# Autodesk Inventor assembly: ASY MSC 500 BELLY
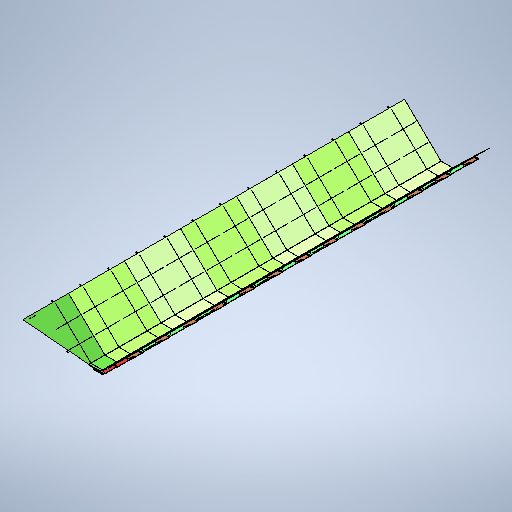
[picture p0: Inventor's stored thumbnail of the model, 512x512]
Saved by Autodesk Inventor 2025 (Build 290162010, 162A)
## iProperties
Created: 2024-07-22
Part Number: ASY MSC 500 BELLY
Document SubType Name: Assembly
Designer: pokla
Stock Number: ASY МОО 500 брюхо
Author: pokla
## Documents named in this file (7)
- C:\Users\admin\YandexDisk-badmisterfox\домашниий пк\Inventor\Manturovo\Manturovo_Se-clar\ASY MSC 204 BELLY.iam
- C:\Users\admin\YandexDisk-badmisterfox\домашниий пк\Inventor\Manturovo\Manturovo_Se-clar\MSC 501 sheet belly main.ipt
- C:\Users\admin\YandexDisk-badmisterfox\домашниий пк\Inventor\Manturovo\Manturovo_Se-clar\MSC 502 sheet belly-neck.ipt
- C:\Users\admin\YandexDisk-badmisterfox\домашниий пк\Inventor\Manturovo\Manturovo_Se-clar\MSC 504 stringer board belly.ipt
- C:\Users\admin\YandexDisk-badmisterfox\домашниий пк\Inventor\Manturovo\Manturovo_Se-clar\MSC 503 rib belly.ipt
- C:\Users\admin\YandexDisk-badmisterfox\домашниий пк\Inventor\Manturovo\Manturovo_Se-clar\MSC 505 sheet belly-neck.ipt
- C:\Users\admin\YandexDisk-badmisterfox\домашниий пк\Inventor\Manturovo\Manturovo_Se-clar\MSC 506 stringer belly short.ipt
## Components (62 placed, 7 different names)
1. MSC 501 sheet belly main:1
2. MSC 501 sheet belly main:2
3. MSC 501 sheet belly main:3
4. MSC 502 sheet belly-neck:1 — Rigid:24
5. MSC 501 sheet belly main:4
6. MSC 501 sheet belly main:5 — Rigid:23, Rigid:24
7. MSC 501 sheet belly main:6 — Mate:4, Mate:5, Mate:6, Mate:7, Flush:1, Mate:9, Mate:10, Flush:2, Mate:11, Mate:12
8. MSC 503 rib belly:1 — Rigid:17, Rigid:20, Rigid:21, Mate:13
9. MSC 503 rib belly:2 — Rigid:18, Rigid:19, Mate:11, Mate:12, Mate:13
10. MSC 504 stringer board belly:1 — Rigid:21, Flush:2
11. MSC 504 stringer board belly:2 — Rigid:20
12. MSC 504 stringer board belly:3 — Rigid:19
13. MSC 504 stringer board belly:4 — Rigid:18
14. MSC 505 sheet belly-neck:1 — Rigid:23
15. MSC 506 stringer belly short:1 — Rigid:25
16. MSC 506 stringer belly short:2 — Rigid:26
17. MSC 506 stringer belly short:3 — Rigid:27
18. MSC 506 stringer belly short:4 — Rigid:28
19. MSC 504 stringer board belly:5
20. MSC 504 stringer board belly:6
21. MSC 504 stringer board belly:7
22. MSC 504 stringer board belly:8
23. MSC 504 stringer board belly:9
24. MSC 504 stringer board belly:10
25. MSC 504 stringer board belly:11
26. MSC 504 stringer board belly:12
27. MSC 504 stringer board belly:13
28. MSC 504 stringer board belly:14
29. MSC 504 stringer board belly:15
30. MSC 504 stringer board belly:16
31. MSC 504 stringer board belly:17
32. MSC 504 stringer board belly:18
33. MSC 504 stringer board belly:19
34. MSC 504 stringer board belly:20
35. MSC 504 stringer board belly:21 — Rigid:28
36. MSC 504 stringer board belly:22 — Rigid:27
37. MSC 504 stringer board belly:23 — Rigid:25
38. MSC 504 stringer board belly:24 — Rigid:26
39. MSC 503 rib belly:3 — Mate:6, Mate:7, Mate:8, Rigid:17
40. MSC 503 rib belly:4 — Mate:4, Mate:5, Mate:8
41. МОО 042 шпангоут брюхо:6
42. МОО 042 шпангоут брюхо:7
43. МОО 042 шпангоут брюхо:8
44. МОО 042 шпангоут брюхо:9
45. МОО 042 шпангоут брюхо:10
46. МОО 042 шпангоут брюхо:11
47. МОО 042 шпангоут брюхо:12
48. МОО 042 шпангоут брюхо:13
49. МОО 042 шпангоут брюхо:14
50. МОО 042 шпангоут брюхо:15
51. МОО 042 шпангоут брюхо:16
52. МОО 042 шпангоут брюхо:17
53. МОО 042 шпангоут брюхо:18
54. МОО 042 шпангоут брюхо:19
55. МОО 042 шпангоут брюхо:20
56. МОО 042 шпангоут брюхо:21
57. МОО 042 шпангоут брюхо:22
58. МОО 042 шпангоут брюхо:23
59. МОО 042 шпангоут брюхо:24
60. МОО 042 шпангоут брюхо:25
61. МОО 042 шпангоут брюхо:26
62. МОО 042 шпангоут брюхо:27
## Component patterns: (5 elements, first: MSC 504 stringer board belly:5 + MSC 504 stringer board belly:6 + MSC 504 stringer board belly:7 + MSC 504 stringer board belly:8), (12 elements, first: MSC 503 rib belly:3 + MSC 503 rib belly:4)
## Relationships (32: WeldJoint 20, Mate 10, Flush 2)
- [WeldJoint]: MSC 501 sheet belly main:1 ↔ MSC 501 sheet belly main:2
- [WeldJoint]: MSC 501 sheet belly main:1 ↔ MSC 501 sheet belly main:3
- [WeldJoint]: MSC 501 sheet belly main:4 ↔ MSC 501 sheet belly main:5
- [WeldJoint]: MSC 501 sheet belly main:3 ↔ MSC 501 sheet belly main:4
- [WeldJoint]: MSC 501 sheet belly main:2 ↔ MSC 501 sheet belly main:6
- [WeldJoint]: MSC 504 stringer board belly:3 ↔ MSC 504 stringer board belly:5
- [WeldJoint]: MSC 504 stringer board belly:4 ↔ MSC 504 stringer board belly:6
- [WeldJoint]: MSC 504 stringer board belly:2 ↔ MSC 504 stringer board belly:7
- [WeldJoint]: MSC 504 stringer board belly:1 ↔ MSC 504 stringer board belly:8
- Mate:4: MSC 501 sheet belly main:6 ↔ MSC 503 rib belly:4
- Mate:5: MSC 501 sheet belly main:6 ↔ MSC 503 rib belly:4
- Mate:6: MSC 501 sheet belly main:6 ↔ MSC 503 rib belly:3
- Mate:7: MSC 501 sheet belly main:6 ↔ MSC 503 rib belly:3
- Mate:8: MSC 503 rib belly:3 ↔ MSC 503 rib belly:4
- Flush:1: MSC 501 sheet belly main:6
- Mate:9: MSC 501 sheet belly main:6
- Mate:10: MSC 501 sheet belly main:6
- Rigid:17 [WeldJoint] (490 mm): MSC 503 rib belly:1 ↔ MSC 503 rib belly:3
- Rigid:18 [WeldJoint]: MSC 503 rib belly:2 ↔ MSC 504 stringer board belly:4
- Rigid:19 [WeldJoint]: MSC 503 rib belly:2 ↔ MSC 504 stringer board belly:3
- Rigid:20 [WeldJoint]: MSC 503 rib belly:1 ↔ MSC 504 stringer board belly:2
- Rigid:21 [WeldJoint]: MSC 503 rib belly:1 ↔ MSC 504 stringer board belly:1
- Flush:2: MSC 501 sheet belly main:6 ↔ MSC 504 stringer board belly:1
- Mate:11: MSC 501 sheet belly main:6 ↔ MSC 503 rib belly:2
- Mate:12: MSC 501 sheet belly main:6 ↔ MSC 503 rib belly:2
- Mate:13: MSC 503 rib belly:1 ↔ MSC 503 rib belly:2
- Rigid:23 [WeldJoint]: MSC 501 sheet belly main:5 ↔ MSC 505 sheet belly-neck:1
- Rigid:24 [WeldJoint]: MSC 502 sheet belly-neck:1 ↔ MSC 501 sheet belly main:5
- Rigid:25 [WeldJoint]: MSC 506 stringer belly short:1 ↔ MSC 504 stringer board belly:23
- Rigid:26 [WeldJoint]: MSC 506 stringer belly short:2 ↔ MSC 504 stringer board belly:24
- Rigid:27 [WeldJoint]: MSC 506 stringer belly short:3 ↔ MSC 504 stringer board belly:22
- Rigid:28 [WeldJoint]: MSC 506 stringer belly short:4 ↔ MSC 504 stringer board belly:21
